# Autodesk Inventor assembly: Gripper_Long_Assembly
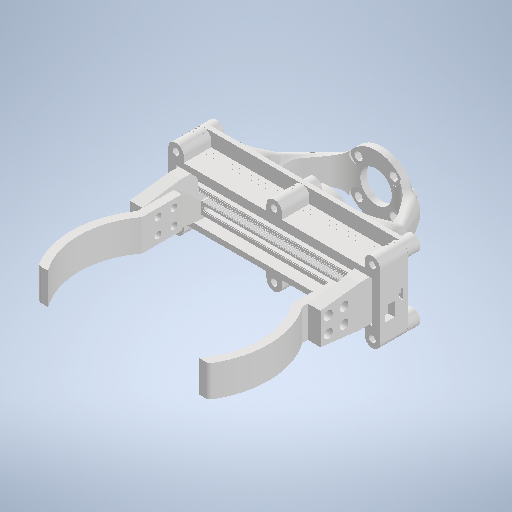
[picture p0: Inventor's stored thumbnail of the model, 512x512]
Saved by Autodesk Inventor 2025.1 (Build 291241000, 241)
## iProperties
Created: 2024-08-03
Part Number: Gripper_Long_Assembly
Document SubType Name: Assembly
Designer: leonh
Mass: 121.571 g
Surface Area: 803.528 cm^2
Volume: 121.571 cm^3
Density: 1 g/cm^3
Author: leonh
## Documents named in this file (7)
- C:\Users\leonh\OneDrive\Dokumente\a_informatik\Inventor\Random\Gripper_Long_Assembly.iam
- C:\Users\leonh\OneDrive\Dokumente\a_informatik\Inventor\Random\Gripper_BackPlate_Long.ipt
- C:\Users\leonh\OneDrive\Dokumente\a_informatik\Inventor\Random\Gripper_Concave_Finger.ipt
- C:\Users\leonh\OneDrive\Dokumente\a_informatik\Inventor\Random\Gripper_Finger_Long.ipt
- C:\Users\leonh\OneDrive\Dokumente\a_informatik\Inventor\Random\Gripper_MountingBlock_Long.ipt
- C:\Users\leonh\OneDrive\Dokumente\a_informatik\Inventor\Random\Gripper_MotorHolder.ipt
- C:\Users\leonh\OneDrive\Dokumente\a_informatik\Inventor\Random\Gripper_FlangeMount.ipt
## Components (8 placed, 6 different names)
1. Gripper_BackPlate_Long:1 — Mate:1, Insert:1, Angle:1, Mate:3, Angle:4, Mate:5, Insert:4
2. Gripper_Concave_Finger:1 — Mate:4, Insert:2, Angle:3
3. Gripper_Finger_Long:1 — Slider:1, Symmetry:1, Insert:3, Angle:2
4. Gripper_MountingBlock_Long:1 — Mate:1, Insert:1, Angle:1, Mate:2
5. Gripper_Finger_Long:2 — Slider:1, Mate:2, Mate:3, Symmetry:1, Mate:4, Insert:2, Angle:3
6. Gripper_Concave_Finger:2 — Insert:3, Angle:2
7. Gripper_MotorHolder:1 — Angle:4, Mate:5, Insert:4, Mate:6, Angle:5, Insert:5
8. Gripper_FlangeMount:1 — Mate:6, Angle:5, Insert:5
## Relationships (18: Mate 6, Insert 5, Angle 5, TranslationJoint 1, Symmetry 1)
- Mate:1: Gripper_BackPlate_Long:1 ↔ Gripper_MountingBlock_Long:1
- Insert:1: Gripper_BackPlate_Long:1 ↔ Gripper_MountingBlock_Long:1
- Slider:1 [TranslationJoint]: Gripper_Finger_Long:1 ↔ Gripper_Finger_Long:2
- Angle:1 (0 deg): Gripper_BackPlate_Long:1 ↔ Gripper_MountingBlock_Long:1
- Mate:2: Gripper_MountingBlock_Long:1 ↔ Gripper_Finger_Long:2
- Mate:3 (0.1 mm): Gripper_BackPlate_Long:1 ↔ Gripper_Finger_Long:2
- Symmetry:1: Gripper_Finger_Long:1 ↔ Gripper_Finger_Long:2
- Mate:4: Gripper_Concave_Finger:1 ↔ Gripper_Finger_Long:2
- Insert:2: Gripper_Concave_Finger:1 ↔ Gripper_Finger_Long:2
- Insert:3: Gripper_Finger_Long:1 ↔ Gripper_Concave_Finger:2
- Angle:2 (0 deg): Gripper_Finger_Long:1 ↔ Gripper_Concave_Finger:2
- Angle:3 (0 deg): Gripper_Concave_Finger:1 ↔ Gripper_Finger_Long:2
- Angle:4 (0 deg): Gripper_BackPlate_Long:1 ↔ Gripper_MotorHolder:1
- Mate:5: Gripper_BackPlate_Long:1 ↔ Gripper_MotorHolder:1
- Insert:4: Gripper_BackPlate_Long:1 ↔ Gripper_MotorHolder:1
- Mate:6: Gripper_MotorHolder:1 ↔ Gripper_FlangeMount:1
- Angle:5 (0 deg): Gripper_MotorHolder:1 ↔ Gripper_FlangeMount:1
- Insert:5: Gripper_MotorHolder:1 ↔ Gripper_FlangeMount:1
